# Autodesk Inventor assembly: toggle switch cover
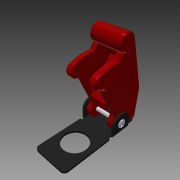
[picture p0: Inventor's stored thumbnail of the model, 180x180]
Saved by Autodesk Inventor 2016 (Build 200138000, 138)
## iProperties
Created: 2014-01-27
Part Number: toggle switch cover
Document SubType Name: Assembly
Designer: Michał
Author: Michał
## Documents named in this file (4)
- C:\Users\agmle\BitTorrent Sync\private\projects\Creekfleet_Timer\hardware\CAD\Main\toggle switch cover.iam
- C:\Users\agmle\BitTorrent Sync\private\projects\Creekfleet_Timer\hardware\CAD\Main\01.ipt
- C:\Users\agmle\BitTorrent Sync\private\projects\Creekfleet_Timer\hardware\CAD\Main\02.ipt
- C:\Users\agmle\BitTorrent Sync\private\projects\Creekfleet_Timer\hardware\CAD\Main\03.ipt
## Components (3 placed, 3 different names)
1. 01:1 — Insert:1, Insert:2
2. 02:1 — Insert:2
3. 03:1 — Insert:1
## Relationships (2: Insert 2)
- Insert:1 (0.25 mm): 01:1 ↔ 03:1
- Insert:2: 01:1 ↔ 02:1
